# Autodesk Inventor assembly: heatSetSampleShowingInserts
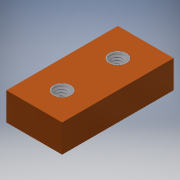
[picture p0: Inventor's stored thumbnail of the model, 180x180]
Saved by Autodesk Inventor 2019.3 (Build 233278000, 278)
## iProperties
Created: 2019-01-12
Part Number: heatSetSampleShowingInserts
Document SubType Name: Assembly
Designer: steele
Author: steele
## Documents named in this file (3)
- C:\git\CAD-Development\robSteele\2019-FRC\heatSetSampleShowingInserts.iam
- C:\git\CAD-Development\robSteele\2019-FRC\seatingPartsExample.ipt
- C:\git\CAD-MfgResources\McMaster-Carr\BrassHeatSetInsertForPlastic\1_4-20 0_375 94459A380_BRASS HEAT-SET INSERT FOR PLASTIC.ipt
## Components (3 placed, 2 different names)
1. seatingPartsExample:1 — Insert:1, Insert:2
2. 1_4-20 0_375 94459A380_BRASS HEAT-SET INSERT FOR PLASTIC:1 — Insert:1
3. 1_4-20 0_375 94459A380_BRASS HEAT-SET INSERT FOR PLASTIC:2 — Insert:2
## Relationships (2: Insert 2)
- Insert:1: seatingPartsExample:1 ↔ 1_4-20 0_375 94459A380_BRASS HEAT-SET INSERT FOR PLASTIC:1
- Insert:2: seatingPartsExample:1 ↔ 1_4-20 0_375 94459A380_BRASS HEAT-SET INSERT FOR PLASTIC:2
